# Autodesk Inventor assembly: Right Claw
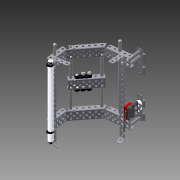
[picture p0: Inventor's stored thumbnail of the model, 180x180]
Saved by Autodesk Inventor 2012 (Build 160160000, 160)
## iProperties
Created: 2011-08-16
Part Number: Right Claw
Document SubType Name: Assembly
Designer: Dakota.Bayer
Author: Dakota.Bayer
## Documents named in this file (27)
- C:\Users\Wade\Documents\1103 Robot - CAD Assembly\Right Claw.iam
- C:\Users\Wade\Documents\1103 Robot - CAD Assembly\2 x 15 bentttttttt.ipt
- C:\Users\Wade\Documents\1103 Robot - CAD Assembly\1 x 20 BENT.ipt
- C:\Users\Wade\Documents\1103 Robot - CAD Assembly\2 x 6 legit.ipt
- C:\Users\Wade\Documents\24C VEX CAD Files\Washers & Spacers\Spacer (Nylon), 0.500''.ipt
- C:\Users\Wade\Documents\24C VEX CAD Files\Other Parts\Shaft Collar (with Set Screw Installed).ipt
- C:\Users\Wade\Documents\24C VEX CAD Files\Standoffs & Couplers\Standoff 2.00''.ipt
- C:\Users\Wade\Documents\24C VEX CAD Files\Standoffs & Couplers\Standoff 5.00''.ipt
- C:\Users\Wade\Documents\24C VEX CAD Files\Standoffs & Couplers\Standoff 1.50''.ipt
- C:\Users\Wade\Documents\24C VEX CAD Files\Washers & Spacers\Spacer (Nylon), 0.125''.ipt
- C:\Users\Wade\Documents\24C VEX CAD Files\Drive Shafts\Drive Shaft (Square Bar) 8''.ipt
- C:\Users\Wade\Documents\24C VEX CAD Files\Washers & Spacers\Spacer (Nylon), 0.250''.ipt
- C:\Users\Wade\Documents\24C VEX CAD Files\Other Parts\(Pillow) Bearing Block mod.ipt
- C:\Users\Wade\Documents\1103 Robot - CAD Assembly\VEX-HINGE-2 RevA_1.ipt
- C:\Users\Wade\Documents\1103 Robot - CAD Assembly\Bearing Assembly (end hole).iam
- C:\Users\Wade\Documents\1103 Robot - CAD Assembly\.375'' Screw & Nylock Nut.iam
- C:\Users\Wade\Documents\24C VEX CAD Files\Screws & Nuts\Screw 8-32 x 0.500''-Silver.ipt
- C:\Users\Wade\Documents\24C VEX CAD Files\Screws & Nuts\Nut 8-32 Nylock.ipt
- C:\Users\Wade\Documents\24C VEX CAD Files\Screws & Nuts\Screw 8-32 x 0.250''-Silver.ipt
- C:\Users\Wade\Documents\24C VEX CAD Files\Standoffs & Couplers\Standoff 1.00''.ipt
- C:\Users\Wade\Documents\24C VEX CAD Files\Metal Angles\Short Slotted Angle (Segmented Angle, 1x1x2).ipt
- C:\Users\Wade\Documents\24C VEX CAD Files\Motors & Sensors\Limit Switch (Sensor).iam
- C:\Users\Wade\Documents\24C VEX CAD Files\Washers & Spacers\Spacer (Thick), 8mm.ipt
- C:\Users\Wade\Documents\24C VEX CAD Files\Screws & Nuts\Screw 8-32 x 0.750''-Silver.ipt
- C:\Users\Wade\Documents\24C VEX CAD Files\Screws & Nuts\Screw 8-32 x 0.625''-Silver.ipt
- C:\Users\Wade\Documents\24C VEX CAD Files\Washers & Spacers\Spacer (Nylon), 0.375''.ipt
- C:\Users\Wade\Documents\24C VEX CAD Files\Screws & Nuts\Screw 8-32 x 1.750''-Silver.ipt
## Components (93 placed, 26 different names)
1. Standoff 1.50'':1 — Mate:803, Mate:805, Mate:852, Mate:856
2. Standoff 1.50'':2 — Mate:804, Mate:853, Mate:857
3. 1 x 20 BENT:1 — Mate:638, Flush:39, Flush:40, Mate:643, Mate:818, Mate:819, Mate:821, Mate:822, Mate:823, Mate:824, Mate:825, Mate:826, Mate:827, Mate:828, Mate:829
4. Standoff 5.00'':1 — Mate:844, Mate:876
5. 2 x 15 bentttttttt:1 — Mate:638, Flush:39, Flush:40, Mate:687, Flush:41, Flush:42, Mate:793, Angle:1, Flush:46, Flush:47, Mate:804, Mate:805, Mate:820, Mate:845, Mate:847, Mate:849, Mate:851, Mate:858, Mate:859, Mate:884, Mate:885, Mate:892, Mate:895
6. 2 x 6 legit:1 — Mate:808, Mate:809, Mate:810, Mate:811, Mate:812, Mate:815, Mate:816, Mate:869, Mate:871, Mate:873, Mate:875
7. 2 x 15 bentttttttt:2 — Mate:643, Mate:795, Mate:796, Mate:797, Flush:48, Mate:862, Mate:863, Mate:877, Mate:879, Mate:881, Mate:883
8. Standoff 5.00'':2 — Mate:850, Mate:882
9. Spacer (Nylon), 0.500'':1
10. Spacer (Nylon), 0.500'':2
11. Spacer (Nylon), 0.500'':3
12. Spacer (Nylon), 0.500'':4
13. Spacer (Nylon), 0.500'':5
14. Spacer (Nylon), 0.500'':6 — Mate:798, Mate:799
15. Spacer (Nylon), 0.500'':7
16. Spacer (Nylon), 0.500'':8
17. Spacer (Nylon), 0.500'':9
18. Spacer (Nylon), 0.500'':10 — Mate:780, Mate:785, Mate:788, Mate:790
19. Spacer (Nylon), 0.500'':11
20. Spacer (Nylon), 0.500'':12
21. Spacer (Nylon), 0.500'':13 — Mate:783, Mate:784
22. Shaft Collar (with Set Screw Installed):1 — Flush:43, Flush:45
23. Shaft Collar (with Set Screw Installed):2 — Mate:785, Flush:44, Mate:789, Angle:1, Angle:2, Flush:45
24. 1 x 20 BENT:2 — Mate:687, Flush:41, Flush:42, Mate:794, Mate:830, Mate:831, Mate:832, Mate:833, Mate:834, Mate:835, Mate:837, Mate:841
25. Standoff 1.50'':3 — Mate:861, Mate:864
26. Standoff 1.50'':4 — Mate:802, Mate:807, Mate:860, Mate:866
27. Standoff 2.00'':1 — Mate:846, Mate:872
28. Standoff 2.00'':2 — Mate:870, Mate:878
29. Standoff 2.00'':3 — Mate:848, Mate:874
30. Standoff 2.00'':4 — Mate:868, Mate:880
31. Spacer (Nylon), 0.125'':1 — Mate:815
32. Spacer (Nylon), 0.125'':2 — Mate:816, Mate:817
33. Drive Shaft (Square Bar) 8'':1 — Mate:780, Flush:43, Flush:44, Angle:2
34. Spacer (Nylon), 0.250'':1 — Mate:783, Mate:784, Mate:801
35. (Pillow) Bearing Block mod:1 — Mate:795, Mate:796, Mate:797, Mate:800, Mate:840, Mate:843
36. (Pillow) Bearing Block mod:2 — Mate:788, Mate:789, Mate:790, Mate:793, Mate:794, Mate:836, Mate:839
37. Spacer (Nylon), 0.250'':2 — Mate:798, Mate:799, Mate:800, Mate:801
38. VEX-HINGE-2 RevA_1:1 — Mate:803, Flush:46, Flush:47, Mate:806, Mate:854, Mate:855
39. VEX-HINGE-2 RevA_1:2 — Mate:802, Mate:806, Mate:807, Flush:48, Mate:865, Mate:867, Flush:50, Mate:896, Mate:930, Mate:931
40. Bearing Assembly (end hole):1 [sub-assembly] — Mate:808, Mate:809, Mate:810, Mate:811, Mate:813, Mate:814, Mate:817, Mate:932, Mate:935
41. Bearing Assembly (end hole):2 [sub-assembly] — Mate:812, Mate:813, Mate:814, Mate:934
42. .375'' Screw & Nylock Nut:1 [sub-assembly] — Mate:819, Mate:820, Mate:821
43. .375'' Screw & Nylock Nut:2 [sub-assembly] — Mate:818, Mate:822, Mate:823
44. .375'' Screw & Nylock Nut:3 [sub-assembly] — Mate:824, Mate:826, Mate:827
45. .375'' Screw & Nylock Nut:4 [sub-assembly] — Mate:825, Mate:828, Mate:829
46. .375'' Screw & Nylock Nut:5 [sub-assembly] — Mate:833, Mate:834, Mate:835
47. .375'' Screw & Nylock Nut:6 [sub-assembly] — Mate:830, Mate:831, Mate:832
48. Screw 8-32 x 0.500''-Silver:1 — Mate:836, Mate:837, Mate:838
49. Nut 8-32 Nylock:1 — Mate:838, Mate:839
50. Screw 8-32 x 0.500''-Silver:2 — Mate:840, Mate:841, Mate:842
51. Nut 8-32 Nylock:2 — Mate:842, Mate:843
52. Screw 8-32 x 0.250''-Silver:1 — Mate:844, Mate:845, Mate:886
53. Screw 8-32 x 0.250''-Silver:2 — Mate:846, Mate:847
54. Screw 8-32 x 0.250''-Silver:3 — Mate:848, Mate:849
55. Screw 8-32 x 0.250''-Silver:4 — Mate:850, Mate:851, Mate:893
56. Screw 8-32 x 0.250''-Silver:5 — Mate:852, Mate:855
57. Screw 8-32 x 0.250''-Silver:6 — Mate:853, Mate:854
58. Screw 8-32 x 0.250''-Silver:7 — Mate:856, Mate:859
59. Screw 8-32 x 0.250''-Silver:8 — Mate:857, Mate:858
60. Screw 8-32 x 0.250''-Silver:9 — Mate:860, Mate:862
61. Screw 8-32 x 0.250''-Silver:10 — Mate:861, Mate:863
62. Screw 8-32 x 0.250''-Silver:11 — Mate:864, Mate:865
63. Screw 8-32 x 0.250''-Silver:12 — Mate:866, Mate:867
64. Screw 8-32 x 0.250''-Silver:13 — Mate:870, Mate:871
65. Screw 8-32 x 0.250''-Silver:14 — Mate:868, Mate:869
66. Screw 8-32 x 0.250''-Silver:15 — Mate:872, Mate:873
67. Screw 8-32 x 0.250''-Silver:16 — Mate:874, Mate:875
68. Screw 8-32 x 0.250''-Silver:17 — Mate:878, Mate:879
69. Screw 8-32 x 0.250''-Silver:18 — Mate:876, Mate:877
70. Screw 8-32 x 0.250''-Silver:19 — Mate:880, Mate:881
71. Screw 8-32 x 0.250''-Silver:20 — Mate:882, Mate:883
72. Standoff 1.00'':1 — Mate:884, Mate:889, Mate:890, Mate:893, Mate:894
73. Standoff 1.00'':2 — Mate:885, Mate:886, Mate:887, Mate:888, Mate:891
74. Screw 8-32 x 0.250''-Silver:21 — Mate:889, Mate:890
75. Screw 8-32 x 0.250''-Silver:22 — Mate:887, Mate:888
76. Screw 8-32 x 0.250''-Silver:23 — Mate:891, Mate:892
77. Screw 8-32 x 0.250''-Silver:24 — Mate:894, Mate:895
78. Short Slotted Angle (Segmented Angle, 1x1x2):1 — Flush:50, Mate:896, Mate:910, Mate:911, Mate:912, Mate:913, Angle:3, Mate:924, Mate:925, Mate:926, Mate:927
79. Limit Switch (Sensor):1 [sub-assembly] — Mate:914, Mate:915, Mate:916, Angle:3, Mate:917, Mate:918, Mate:920, Mate:921
80. Screw 8-32 x 0.625''-Silver:1 — Mate:928
81. Screw 8-32 x 0.625''-Silver:2 — Mate:929
82. Spacer (Thick), 8mm:1 — Mate:911, Mate:912, Mate:915, Mate:916
83. Spacer (Thick), 8mm:2 — Mate:910, Mate:913, Mate:914, Mate:917, Mate:919
84. Nut 8-32 Nylock:3 — Mate:922, Mate:925
85. Screw 8-32 x 0.750''-Silver:1 — Mate:919, Mate:920, Mate:923
86. Nut 8-32 Nylock:4 — Mate:923, Mate:924
87. Screw 8-32 x 0.750''-Silver:2 — Mate:918, Mate:921, Mate:922
88. Spacer (Nylon), 0.375'':2 — Mate:926
89. Spacer (Nylon), 0.375'':1 — Mate:927
90. Nut 8-32 Nylock:5 — Mate:928, Mate:931
91. Nut 8-32 Nylock:6 — Mate:929, Mate:930
92. Nut 8-32 Nylock:7 — Mate:933, Mate:934
93. Screw 8-32 x 1.750''-Silver:1 — Mate:932, Mate:933, Mate:935
## Relationships (224: Mate 185, Tangent 25, Flush 11, Angle 3)
- [Mate]: Standoff 1.50'':1 ↔ 2 x 15 bentttttttt:1
- [Tangent] (0.2286 mm): Standoff 1.50'':2 ↔ 2 x 15 bentttttttt:1
- [Tangent] (0.2286 mm): Standoff 1.50'':2 ↔ 2 x 15 bentttttttt:1
- [Tangent] (0.2286 mm): Standoff 1.50'':1 ↔ 2 x 15 bentttttttt:1
- Mate:638: 1 x 20 BENT:1 ↔ 2 x 15 bentttttttt:1
- Flush:39: 1 x 20 BENT:1 ↔ 2 x 15 bentttttttt:1
- Flush:40: 1 x 20 BENT:1 ↔ 2 x 15 bentttttttt:1
- [Mate]: Standoff 5.00'':1 ↔ 2 x 15 bentttttttt:2
- Mate:643: 1 x 20 BENT:1 ↔ 2 x 15 bentttttttt:2
- [Tangent] (0.2286 mm): Standoff 5.00'':1 ↔ 2 x 15 bentttttttt:2
- [Tangent] (0.2286 mm): Standoff 5.00'':1 ↔ 2 x 15 bentttttttt:2
- [Mate]: Standoff 5.00'':1 ↔ 2 x 15 bentttttttt:1
- [Tangent] (0.2286 mm): Standoff 5.00'':1 ↔ 2 x 15 bentttttttt:1
- [Tangent] (0.2286 mm): Standoff 5.00'':1 ↔ 2 x 15 bentttttttt:1
- [Mate]: 2 x 15 bentttttttt:1 ↔ Standoff 5.00'':2
- [Tangent] (0.2286 mm): 2 x 15 bentttttttt:1 ↔ Standoff 5.00'':2
- [Tangent] (0.2286 mm): 2 x 15 bentttttttt:1 ↔ Standoff 5.00'':2
- [Mate]: Spacer (Nylon), 0.500'':10 ↔ Spacer (Nylon), 0.500'':12
- [Mate]: Spacer (Nylon), 0.500'':6 ↔ Spacer (Nylon), 0.500'':7
- [Mate]: Spacer (Nylon), 0.500'':1 ↔ Spacer (Nylon), 0.500'':5
- [Mate]: Spacer (Nylon), 0.500'':5 ↔ Spacer (Nylon), 0.500'':7
- [Mate]: Spacer (Nylon), 0.500'':4 ↔ Spacer (Nylon), 0.500'':8
- [Mate]: Spacer (Nylon), 0.500'':2 ↔ Spacer (Nylon), 0.500'':3
- [Mate]: Spacer (Nylon), 0.500'':2 ↔ Spacer (Nylon), 0.500'':4
- [Mate]: Spacer (Nylon), 0.500'':6 ↔ Spacer (Nylon), 0.500'':7
- [Mate]: Spacer (Nylon), 0.500'':5 ↔ Spacer (Nylon), 0.500'':7
- [Mate]: Spacer (Nylon), 0.500'':1 ↔ Spacer (Nylon), 0.500'':5
- [Mate]: Spacer (Nylon), 0.500'':2 ↔ Spacer (Nylon), 0.500'':3
- [Mate]: Spacer (Nylon), 0.500'':2 ↔ Spacer (Nylon), 0.500'':4
- [Mate]: Spacer (Nylon), 0.500'':4 ↔ Spacer (Nylon), 0.500'':8
- [Mate]: Spacer (Nylon), 0.500'':1 ↔ Spacer (Nylon), 0.500'':3
- [Mate]: Spacer (Nylon), 0.500'':1 ↔ Spacer (Nylon), 0.500'':3
- [Mate]: Spacer (Nylon), 0.500'':10 ↔ Spacer (Nylon), 0.500'':12
- [Mate]: Spacer (Nylon), 0.500'':9 ↔ Spacer (Nylon), 0.500'':12
- [Mate]: Spacer (Nylon), 0.500'':9 ↔ Spacer (Nylon), 0.500'':11
- [Mate]: Spacer (Nylon), 0.500'':9 ↔ Spacer (Nylon), 0.500'':11
- [Mate]: Spacer (Nylon), 0.500'':9 ↔ Spacer (Nylon), 0.500'':12
- [Mate]: Spacer (Nylon), 0.500'':9 ↔ Spacer (Nylon), 0.500'':11
- [Mate]: Spacer (Nylon), 0.500'':9 ↔ Spacer (Nylon), 0.500'':12
- [Mate]: Spacer (Nylon), 0.500'':8 ↔ Spacer (Nylon), 0.500'':11
- [Mate]: Spacer (Nylon), 0.500'':8 ↔ Spacer (Nylon), 0.500'':11
- [Mate]: Spacer (Nylon), 0.500'':13 ↔ Shaft Collar (with Set Screw Installed):1
- [Mate]: Spacer (Nylon), 0.500'':13 ↔ Shaft Collar (with Set Screw Installed):1
- Mate:687: 2 x 15 bentttttttt:1 ↔ 1 x 20 BENT:2
- Flush:41: 2 x 15 bentttttttt:1 ↔ 1 x 20 BENT:2
- Flush:42: 2 x 15 bentttttttt:1 ↔ 1 x 20 BENT:2
- [Mate]: 2 x 15 bentttttttt:2 ↔ Standoff 1.50'':3
- [Mate]: 2 x 15 bentttttttt:2 ↔ Standoff 1.50'':4
- [Tangent] (0.2286 mm): 2 x 15 bentttttttt:2 ↔ Standoff 1.50'':4
- [Tangent] (0.2286 mm): 2 x 15 bentttttttt:2 ↔ Standoff 1.50'':4
- [Tangent] (0.2286 mm): 2 x 15 bentttttttt:2 ↔ Standoff 1.50'':3
- [Tangent] (0.2286 mm): 2 x 15 bentttttttt:2 ↔ Standoff 1.50'':3
- [Mate]: 2 x 15 bentttttttt:1 ↔ Standoff 2.00'':1
- [Mate]: 2 x 6 legit:1 ↔ Standoff 2.00'':1
- [Mate]: 2 x 6 legit:1 ↔ Standoff 2.00'':2
- [Tangent] (0.2286 mm): 2 x 15 bentttttttt:1 ↔ Standoff 2.00'':1
- [Tangent] (0.2286 mm): 2 x 15 bentttttttt:1 ↔ Standoff 2.00'':1
- [Tangent] (0.2286 mm): 2 x 6 legit:1 ↔ Standoff 2.00'':1
- [Tangent] (0.2286 mm): 2 x 6 legit:1 ↔ Standoff 2.00'':1
- [Tangent] (0.2286 mm): 2 x 6 legit:1 ↔ Standoff 2.00'':2
- [Tangent] (0.2286 mm): 2 x 6 legit:1 ↔ Standoff 2.00'':2
- [Mate]: 2 x 15 bentttttttt:1 ↔ Standoff 2.00'':3
- [Tangent] (0.2286 mm): 2 x 15 bentttttttt:1 ↔ Standoff 2.00'':3
- [Tangent] (0.2286 mm): 2 x 15 bentttttttt:1 ↔ Standoff 2.00'':3
- [Tangent] (0.2286 mm): 2 x 6 legit:1 ↔ Standoff 2.00'':3
- [Tangent] (0.2286 mm): 2 x 6 legit:1 ↔ Standoff 2.00'':3
- [Mate]: 2 x 6 legit:1 ↔ Standoff 2.00'':4
- [Tangent] (0.2286 mm): 2 x 6 legit:1 ↔ Standoff 2.00'':4
- [Tangent] (0.2286 mm): 2 x 6 legit:1 ↔ Standoff 2.00'':4
- [Mate]: Spacer (Nylon), 0.125'':1 ↔ Spacer (Nylon), 0.125'':2
- Mate:780: Spacer (Nylon), 0.500'':10 ↔ Drive Shaft (Square Bar) 8'':1
- Mate:783: Spacer (Nylon), 0.500'':13 ↔ Spacer (Nylon), 0.250'':1
- Mate:784: Spacer (Nylon), 0.500'':13 ↔ Spacer (Nylon), 0.250'':1
- Flush:43: Shaft Collar (with Set Screw Installed):1 ↔ Drive Shaft (Square Bar) 8'':1
- Mate:785: Spacer (Nylon), 0.500'':10 ↔ Shaft Collar (with Set Screw Installed):2
- Flush:44: Shaft Collar (with Set Screw Installed):2 ↔ Drive Shaft (Square Bar) 8'':1
- Mate:788: Spacer (Nylon), 0.500'':10 ↔ (Pillow) Bearing Block mod:2
- Mate:789 (3.175 mm): Shaft Collar (with Set Screw Installed):2 ↔ (Pillow) Bearing Block mod:2
- Mate:790 (3.175 mm): Spacer (Nylon), 0.500'':10 ↔ (Pillow) Bearing Block mod:2
- Mate:793 (2.3114 mm): 2 x 15 bentttttttt:1 ↔ (Pillow) Bearing Block mod:2
- Mate:794 (2.3114 mm): 1 x 20 BENT:2 ↔ (Pillow) Bearing Block mod:2
- Mate:795 (2.3114 mm): 2 x 15 bentttttttt:2 ↔ (Pillow) Bearing Block mod:1
- Mate:796: 2 x 15 bentttttttt:2 ↔ (Pillow) Bearing Block mod:1
- Mate:797 (2.3114 mm): 2 x 15 bentttttttt:2 ↔ (Pillow) Bearing Block mod:1
- Angle:1 (0 deg): 2 x 15 bentttttttt:1 ↔ Shaft Collar (with Set Screw Installed):2
- Angle:2 (0 deg): Shaft Collar (with Set Screw Installed):2 ↔ Drive Shaft (Square Bar) 8'':1
- Flush:45: Shaft Collar (with Set Screw Installed):1 ↔ Shaft Collar (with Set Screw Installed):2
- Mate:798: Spacer (Nylon), 0.500'':6 ↔ Spacer (Nylon), 0.250'':2
- Mate:799: Spacer (Nylon), 0.500'':6 ↔ Spacer (Nylon), 0.250'':2
- Mate:800: (Pillow) Bearing Block mod:1 ↔ Spacer (Nylon), 0.250'':2
- Mate:801: Spacer (Nylon), 0.250'':1 ↔ Spacer (Nylon), 0.250'':2
- Mate:802: Standoff 1.50'':4 ↔ VEX-HINGE-2 RevA_1:2
- Mate:803: Standoff 1.50'':1 ↔ VEX-HINGE-2 RevA_1:1
- Flush:46: 2 x 15 bentttttttt:1 ↔ VEX-HINGE-2 RevA_1:1
- Flush:47: 2 x 15 bentttttttt:1 ↔ VEX-HINGE-2 RevA_1:1
- Mate:804: Standoff 1.50'':2 ↔ 2 x 15 bentttttttt:1
- Mate:805 (2.3114 mm): Standoff 1.50'':1 ↔ 2 x 15 bentttttttt:1
- Mate:806: VEX-HINGE-2 RevA_1:1 ↔ VEX-HINGE-2 RevA_1:2
- Mate:807: Standoff 1.50'':4 ↔ VEX-HINGE-2 RevA_1:2
- Flush:48: 2 x 15 bentttttttt:2 ↔ VEX-HINGE-2 RevA_1:2
- Mate:808: 2 x 6 legit:1 ↔ Bearing Assembly (end hole):1
- Mate:809 (2.3114 mm): 2 x 6 legit:1 ↔ Bearing Assembly (end hole):1
- Mate:810 (2.3114 mm): 2 x 6 legit:1 ↔ Bearing Assembly (end hole):1
- Mate:811 (2.3114 mm): 2 x 6 legit:1 ↔ Bearing Assembly (end hole):1
- Mate:812: 2 x 6 legit:1 ↔ Bearing Assembly (end hole):2
- Mate:813: Bearing Assembly (end hole):1 ↔ Bearing Assembly (end hole):2
- Mate:814: Bearing Assembly (end hole):1 ↔ Bearing Assembly (end hole):2
- Mate:815: 2 x 6 legit:1 ↔ Spacer (Nylon), 0.125'':1
- Mate:816: 2 x 6 legit:1 ↔ Spacer (Nylon), 0.125'':2
- Mate:817: Spacer (Nylon), 0.125'':2 ↔ Bearing Assembly (end hole):1
- Mate:818: 1 x 20 BENT:1 ↔ .375'' Screw & Nylock Nut:2
- Mate:819: 1 x 20 BENT:1 ↔ .375'' Screw & Nylock Nut:1
- Mate:820 (2.3114 mm): 2 x 15 bentttttttt:1 ↔ .375'' Screw & Nylock Nut:1
- Mate:821 (2.3114 mm): 1 x 20 BENT:1 ↔ .375'' Screw & Nylock Nut:1
- Mate:822 (2.3114 mm): 1 x 20 BENT:1 ↔ .375'' Screw & Nylock Nut:2
- Mate:823 (2.3114 mm): 1 x 20 BENT:1 ↔ .375'' Screw & Nylock Nut:2
- Mate:824: 1 x 20 BENT:1 ↔ .375'' Screw & Nylock Nut:3
- Mate:825: 1 x 20 BENT:1 ↔ .375'' Screw & Nylock Nut:4
- Mate:826 (2.3114 mm): 1 x 20 BENT:1 ↔ .375'' Screw & Nylock Nut:3
- Mate:827 (2.3114 mm): 1 x 20 BENT:1 ↔ .375'' Screw & Nylock Nut:3
- Mate:828 (2.3114 mm): 1 x 20 BENT:1 ↔ .375'' Screw & Nylock Nut:4
- Mate:829 (2.3114 mm): 1 x 20 BENT:1 ↔ .375'' Screw & Nylock Nut:4
- Mate:830: 1 x 20 BENT:2 ↔ .375'' Screw & Nylock Nut:6
- Mate:831 (2.3114 mm): 1 x 20 BENT:2 ↔ .375'' Screw & Nylock Nut:6
- Mate:832 (2.3114 mm): 1 x 20 BENT:2 ↔ .375'' Screw & Nylock Nut:6
- Mate:833: 1 x 20 BENT:2 ↔ .375'' Screw & Nylock Nut:5
- Mate:834 (2.3114 mm): 1 x 20 BENT:2 ↔ .375'' Screw & Nylock Nut:5
- Mate:835 (2.3114 mm): 1 x 20 BENT:2 ↔ .375'' Screw & Nylock Nut:5
- Mate:836: (Pillow) Bearing Block mod:2 ↔ Screw 8-32 x 0.500''-Silver:1
- Mate:837: 1 x 20 BENT:2 ↔ Screw 8-32 x 0.500''-Silver:1
- Mate:838: Screw 8-32 x 0.500''-Silver:1 ↔ Nut 8-32 Nylock:1
- Mate:839: (Pillow) Bearing Block mod:2 ↔ Nut 8-32 Nylock:1
- Mate:840: (Pillow) Bearing Block mod:1 ↔ Screw 8-32 x 0.500''-Silver:2
- Mate:841: 1 x 20 BENT:2 ↔ Screw 8-32 x 0.500''-Silver:2
- Mate:842: Screw 8-32 x 0.500''-Silver:2 ↔ Nut 8-32 Nylock:2
- Mate:843: (Pillow) Bearing Block mod:1 ↔ Nut 8-32 Nylock:2
- Mate:844: Standoff 5.00'':1 ↔ Screw 8-32 x 0.250''-Silver:1
- Mate:845: 2 x 15 bentttttttt:1 ↔ Screw 8-32 x 0.250''-Silver:1
- Mate:846: Standoff 2.00'':1 ↔ Screw 8-32 x 0.250''-Silver:2
- Mate:847: 2 x 15 bentttttttt:1 ↔ Screw 8-32 x 0.250''-Silver:2
- Mate:848: Standoff 2.00'':3 ↔ Screw 8-32 x 0.250''-Silver:3
- Mate:849: 2 x 15 bentttttttt:1 ↔ Screw 8-32 x 0.250''-Silver:3
- Mate:850: Standoff 5.00'':2 ↔ Screw 8-32 x 0.250''-Silver:4
- Mate:851: 2 x 15 bentttttttt:1 ↔ Screw 8-32 x 0.250''-Silver:4
- Mate:852: Standoff 1.50'':1 ↔ Screw 8-32 x 0.250''-Silver:5
- Mate:853: Standoff 1.50'':2 ↔ Screw 8-32 x 0.250''-Silver:6
- Mate:854: VEX-HINGE-2 RevA_1:1 ↔ Screw 8-32 x 0.250''-Silver:6
- Mate:855: VEX-HINGE-2 RevA_1:1 ↔ Screw 8-32 x 0.250''-Silver:5
- Mate:856: Standoff 1.50'':1 ↔ Screw 8-32 x 0.250''-Silver:7
- Mate:857: Standoff 1.50'':2 ↔ Screw 8-32 x 0.250''-Silver:8
- Mate:858: 2 x 15 bentttttttt:1 ↔ Screw 8-32 x 0.250''-Silver:8
- Mate:859: 2 x 15 bentttttttt:1 ↔ Screw 8-32 x 0.250''-Silver:7
- Mate:860: Standoff 1.50'':4 ↔ Screw 8-32 x 0.250''-Silver:9
- Mate:861: Standoff 1.50'':3 ↔ Screw 8-32 x 0.250''-Silver:10
- Mate:862: 2 x 15 bentttttttt:2 ↔ Screw 8-32 x 0.250''-Silver:9
- Mate:863: 2 x 15 bentttttttt:2 ↔ Screw 8-32 x 0.250''-Silver:10
- Mate:864: Standoff 1.50'':3 ↔ Screw 8-32 x 0.250''-Silver:11
- Mate:865: VEX-HINGE-2 RevA_1:2 ↔ Screw 8-32 x 0.250''-Silver:11
- Mate:866: Standoff 1.50'':4 ↔ Screw 8-32 x 0.250''-Silver:12
- Mate:867: VEX-HINGE-2 RevA_1:2 ↔ Screw 8-32 x 0.250''-Silver:12
- Mate:868: Standoff 2.00'':4 ↔ Screw 8-32 x 0.250''-Silver:14
- Mate:869: 2 x 6 legit:1 ↔ Screw 8-32 x 0.250''-Silver:14
- Mate:870: Standoff 2.00'':2 ↔ Screw 8-32 x 0.250''-Silver:13
- Mate:871: 2 x 6 legit:1 ↔ Screw 8-32 x 0.250''-Silver:13
- Mate:872: Standoff 2.00'':1 ↔ Screw 8-32 x 0.250''-Silver:15
- Mate:873: 2 x 6 legit:1 ↔ Screw 8-32 x 0.250''-Silver:15
- Mate:874: Standoff 2.00'':3 ↔ Screw 8-32 x 0.250''-Silver:16
- Mate:875: 2 x 6 legit:1 ↔ Screw 8-32 x 0.250''-Silver:16
- Mate:876: Standoff 5.00'':1 ↔ Screw 8-32 x 0.250''-Silver:18
- Mate:877: 2 x 15 bentttttttt:2 ↔ Screw 8-32 x 0.250''-Silver:18
- Mate:878: Standoff 2.00'':2 ↔ Screw 8-32 x 0.250''-Silver:17
- Mate:879: 2 x 15 bentttttttt:2 ↔ Screw 8-32 x 0.250''-Silver:17
- Mate:880: Standoff 2.00'':4 ↔ Screw 8-32 x 0.250''-Silver:19
- Mate:881: 2 x 15 bentttttttt:2 ↔ Screw 8-32 x 0.250''-Silver:19
- Mate:882: Standoff 5.00'':2 ↔ Screw 8-32 x 0.250''-Silver:20
- Mate:883: 2 x 15 bentttttttt:2 ↔ Screw 8-32 x 0.250''-Silver:20
- Mate:884: 2 x 15 bentttttttt:1 ↔ Standoff 1.00'':1
- Mate:885: 2 x 15 bentttttttt:1 ↔ Standoff 1.00'':2
- Mate:886: Screw 8-32 x 0.250''-Silver:1 ↔ Standoff 1.00'':2
- Mate:887: Standoff 1.00'':2 ↔ Screw 8-32 x 0.250''-Silver:22
- Mate:888: Standoff 1.00'':2 ↔ Screw 8-32 x 0.250''-Silver:22
- Mate:889: Standoff 1.00'':1 ↔ Screw 8-32 x 0.250''-Silver:21
- Mate:890: Standoff 1.00'':1 ↔ Screw 8-32 x 0.250''-Silver:21
- Mate:891: Standoff 1.00'':2 ↔ Screw 8-32 x 0.250''-Silver:23
- Mate:892: 2 x 15 bentttttttt:1 ↔ Screw 8-32 x 0.250''-Silver:23
- Mate:893: Screw 8-32 x 0.250''-Silver:4 ↔ Standoff 1.00'':1
- Mate:894: Standoff 1.00'':1 ↔ Screw 8-32 x 0.250''-Silver:24
- Mate:895: 2 x 15 bentttttttt:1 ↔ Screw 8-32 x 0.250''-Silver:24
- Flush:50: VEX-HINGE-2 RevA_1:2 ↔ Short Slotted Angle (Segmented Angle, 1x1x2):1
- Mate:896 (9.5377 mm): VEX-HINGE-2 RevA_1:2 ↔ Short Slotted Angle (Segmented Angle, 1x1x2):1
- [Mate]: Short Slotted Angle (Segmented Angle, 1x1x2):1 ↔ Spacer (Nylon), 0.375'':2
- [Mate]: Short Slotted Angle (Segmented Angle, 1x1x2):1 ↔ Spacer (Nylon), 0.375'':1
- [Mate]: Screw 8-32 x 0.625''-Silver:1 ↔ Spacer (Nylon), 0.375'':1
- [Mate]: Screw 8-32 x 0.625''-Silver:2 ↔ Spacer (Nylon), 0.375'':2
- [Mate]: Short Slotted Angle (Segmented Angle, 1x1x2):1 ↔ Screw 8-32 x 0.625''-Silver:1
- [Mate]: Short Slotted Angle (Segmented Angle, 1x1x2):1 ↔ Screw 8-32 x 0.625''-Silver:2
- [Mate] (2.3114 mm): VEX-HINGE-2 RevA_1:2 ↔ Spacer (Nylon), 0.375'':2
- Mate:910: Short Slotted Angle (Segmented Angle, 1x1x2):1 ↔ Spacer (Thick), 8mm:2
- Mate:911: Short Slotted Angle (Segmented Angle, 1x1x2):1 ↔ Spacer (Thick), 8mm:1
- Mate:912: Short Slotted Angle (Segmented Angle, 1x1x2):1 ↔ Spacer (Thick), 8mm:1
- Mate:913: Short Slotted Angle (Segmented Angle, 1x1x2):1 ↔ Spacer (Thick), 8mm:2
- Mate:914 (2.2225 mm): Limit Switch (Sensor):1 ↔ Spacer (Thick), 8mm:2
- Mate:915 (2.2225 mm): Limit Switch (Sensor):1 ↔ Spacer (Thick), 8mm:1
- Mate:916: Limit Switch (Sensor):1 ↔ Spacer (Thick), 8mm:1
- Angle:3 (0 deg): Short Slotted Angle (Segmented Angle, 1x1x2):1 ↔ Limit Switch (Sensor):1
- Mate:917: Limit Switch (Sensor):1 ↔ Spacer (Thick), 8mm:2
- Mate:918: Limit Switch (Sensor):1 ↔ Screw 8-32 x 0.750''-Silver:2
- Mate:919: Spacer (Thick), 8mm:2 ↔ Screw 8-32 x 0.750''-Silver:1
- Mate:920: Limit Switch (Sensor):1 ↔ Screw 8-32 x 0.750''-Silver:1
- Mate:921: Limit Switch (Sensor):1 ↔ Screw 8-32 x 0.750''-Silver:2
- Mate:922: Nut 8-32 Nylock:3 ↔ Screw 8-32 x 0.750''-Silver:2
- Mate:923: Screw 8-32 x 0.750''-Silver:1 ↔ Nut 8-32 Nylock:4
- Mate:924: Short Slotted Angle (Segmented Angle, 1x1x2):1 ↔ Nut 8-32 Nylock:4
- Mate:925: Short Slotted Angle (Segmented Angle, 1x1x2):1 ↔ Nut 8-32 Nylock:3
- Mate:926: Short Slotted Angle (Segmented Angle, 1x1x2):1 ↔ Spacer (Nylon), 0.375'':2
- Mate:927: Short Slotted Angle (Segmented Angle, 1x1x2):1 ↔ Spacer (Nylon), 0.375'':1
- Mate:928: Screw 8-32 x 0.625''-Silver:1 ↔ Nut 8-32 Nylock:5
- Mate:929: Screw 8-32 x 0.625''-Silver:2 ↔ Nut 8-32 Nylock:6
- Mate:930: VEX-HINGE-2 RevA_1:2 ↔ Nut 8-32 Nylock:6
- Mate:931: VEX-HINGE-2 RevA_1:2 ↔ Nut 8-32 Nylock:5
- Mate:932: Bearing Assembly (end hole):1 ↔ Screw 8-32 x 1.750''-Silver:1
- Mate:933: Nut 8-32 Nylock:7 ↔ Screw 8-32 x 1.750''-Silver:1
- Mate:934: Bearing Assembly (end hole):2 ↔ Nut 8-32 Nylock:7
- Mate:935: Bearing Assembly (end hole):1 ↔ Screw 8-32 x 1.750''-Silver:1
